# Autodesk Inventor assembly: Ensamblaje1
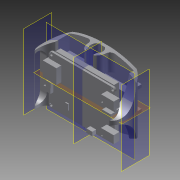
[picture p0: Inventor's stored thumbnail of the model, 180x180]
Saved by Autodesk Inventor 2012 (Build 160160000, 160)
## iProperties
Created: 2012-12-28
Part Number: Ensamblaje1
Document SubType Name: Assembly
Designer: otrebor
Author: otrebor
## Documents named in this file (5)
- C:\Users\otrebor\Desktop\MODI\Ensamblaje1.iam
- C:\Users\otrebor\Desktop\MODI\chasis.ipt
- C:\Users\otrebor\Desktop\MODI\bateria.ipt
- C:\Users\otrebor\Desktop\MODI\fio.ipt
- C:\Users\otrebor\Desktop\MODI\lipoRiderPro.ipt
## Components (4 placed, 4 different names)
1. chasis:1 — Coincidencia:1, Coincidencia:2, Coincidencia:4, Coincidencia:5
2. bateria:1 — Coincidencia:3, Coincidencia:4, Coincidencia:5
3. fio:1 — Coincidencia:1, Coincidencia:2
4. lipoRiderPro:1 — Coincidencia:3
## Relationships (5: Mate 5)
- Coincidencia:1 [Mate]: chasis:1 ↔ fio:1
- Coincidencia:2 [Mate]: chasis:1 ↔ fio:1
- Coincidencia:3 [Mate]: bateria:1 ↔ lipoRiderPro:1
- Coincidencia:4 [Mate]: chasis:1 ↔ bateria:1
- Coincidencia:5 [Mate]: chasis:1 ↔ bateria:1
